# Autodesk Inventor assembly: czlon 1 i 2
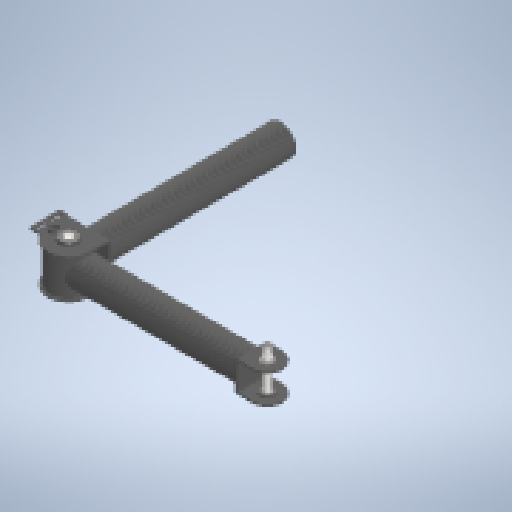
[picture p0: Inventor's stored thumbnail of the model, 512x512]
Saved by Autodesk Inventor 2023 (Build 270158000, 158)
## iProperties
Created: 2023-04-09
Part Number: czlon 1 i 2
Document SubType Name: Assembly
Designer: Wiktor
Mass: 4727.07 g
Surface Area: 10566.9 cm^2
Volume: 2560.65 cm^3
Density: 1.84605 g/cm^3
Author: Wiktor
## Documents named in this file (10)
- C:\Users\krzys\Documents\GitHub\Manipulator-Inventor\czlon 1 i 2.iam
- C:\Users\krzys\Documents\GitHub\Manipulator-Inventor\czlon i przekladnia.iam
- C:\Users\krzys\Documents\GitHub\Manipulator-Inventor\Wał1.ipt
- C:\Users\krzys\Documents\GitHub\Manipulator-Inventor\czlon 2.ipt
- C:\Users\krzys\Documents\GitHub\Manipulator-Inventor\czlon 1 i 2\Design Accelerator\Łożysko2.iam
- C:\Users\krzys\Documents\GitHub\Manipulator-Inventor\Wał3.ipt
- C:\Users\krzys\Documents\GitHub\Manipulator-Inventor\czlon 1 i 2\Design Accelerator\Łożysko3.iam
- C:\Users\krzys\Documents\GitHub\Manipulator-Inventor\czlon 1 i 2\Design Accelerator\Łożysko4.iam
- C:\Users\krzys\Documents\Inventor\Content Center Files\R2023\pl-PL\DIN 933\DIN 933 - M8  x 16.ipt
- C:\Users\krzys\Documents\Inventor\Content Center Files\R2023\pl-PL\DIN 9021\DIN 9021 - 8,4.ipt
## Components (10 placed, 7 different names)
1. czlon i przekladnia:1 [sub-assembly] — Równoległe:1, Wstawiające:5, Wstawiające:6
2. Wał2:1 — Zestawiające:10, Wstawiające:4
3. czlon 2:1 — Zestawiające:10, Równoległe:1, Wstawiające:2, Wstawiające:3
4. Łożysko:4 [sub-assembly] — Wstawiające:3, Zestawiające:11, Równoległe:2, Kątowe:1
5. Łożysko:5 [sub-assembly] — Wstawiające:2
6. Wał3:1 — Zestawiające:11, Równoległe:2, Kątowe:1, Zestawiające:14, Zestawiające:15
7. Łożysko:6 [sub-assembly] — Wstawiające:4, Wstawiające:6
8. Łożysko:7 [sub-assembly] — Wstawiające:5
9. DIN 9021 8,4:1 — Zestawiające:14, Zestawiające:15, Wstawiające:7
10. DIN 933 - zastąpiona przez DIN EN 24017 M8  x 16:1 — Wstawiające:7
## Relationships (13: Insert 6, Mate 4, Flush 2, Angle 1)
- Zestawiające:10 [Mate]: Wał2:1 ↔ czlon 2:1
- Równoległe:1 [Flush]: czlon i przekladnia:1 ↔ czlon 2:1
- Wstawiające:2 [Insert]: czlon 2:1 ↔ Łożysko:5
- Wstawiające:3 [Insert]: czlon 2:1 ↔ Łożysko:4
- Wstawiające:4 [Insert] (-1 mm): Wał2:1 ↔ Łożysko:6
- Wstawiające:5 [Insert] (-1 mm): czlon i przekladnia:1 ↔ Łożysko:7
- Wstawiające:6 [Insert]: czlon i przekladnia:1 ↔ Łożysko:6
- Zestawiające:11 [Mate]: Łożysko:4 ↔ Wał3:1
- Równoległe:2 [Flush]: Łożysko:4 ↔ Wał3:1
- Kątowe:1 [Angle] (0 deg): Łożysko:4 ↔ Wał3:1
- Zestawiające:14 [Mate]: Wał3:1 ↔ DIN 9021 8,4:1
- Zestawiające:15 [Mate]: Wał3:1 ↔ DIN 9021 8,4:1
- Wstawiające:7 [Insert]: DIN 9021 8,4:1 ↔ DIN 933 - zastąpiona przez DIN EN 24017 M8  x 16:1
